# Autodesk Inventor assembly: Wrist
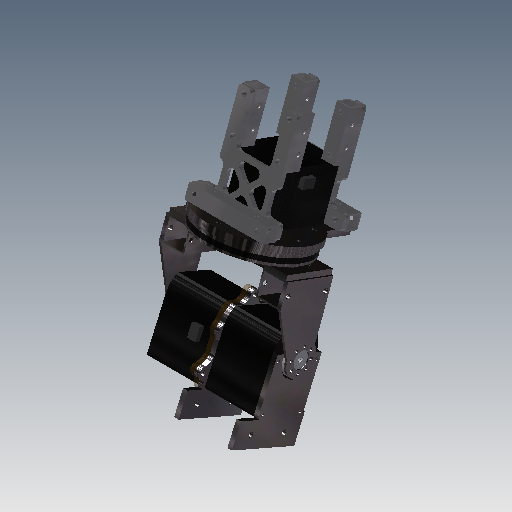
[picture p0: Inventor's stored thumbnail of the model, 512x512]
Saved by Autodesk Inventor 2019.4 (Build 234330000, 330)
## iProperties
Created: 2019-06-30
Part Number: Wrist
Document SubType Name: Assembly
Designer: AzLIer
Author: AzLIer
## Documents named in this file (7)
- E:\ロボ研\キャチロボ\キャチロボ2019\CADdata\アーム2019\Wrist\Wrist.iam
- E:\ロボ研\キャチロボ\キャチロボ2019\CADdata\アーム2019\Wrist\Slide_2_ver2.iam
- E:\ロボ研\キャチロボ\キャチロボ2019\CADdata\アーム2019\Wrist\肩ピッチユニット固定角柱A_9×9.ipt
- E:\ロボ研\キャチロボ\キャチロボ2019\CADdata\アーム2019\Wrist\肩ピッチ固定板_アルミ(A2017)_t3.ipt
- E:\ロボ研\キャチロボ\キャチロボ2019\CADdata\アーム2019\Wrist\肩ピッチ固定角柱B_9×9.ipt
- E:\ロボ研\キャチロボ\キャチロボ2019\CADdata\アーム2019\Wrist\手首関節.iam
- E:\ロボ研\キャチロボ\キャチロボ2019\CADdata\アーム2019\Wrist\先端アームパーツA.ipt
## Components (11 placed, 6 different names)
1. Slide_2:1 [sub-assembly] — 回転:2
2. 肩ピッチユニット固定角柱A_9×9:1
3. 肩ピッチユニット固定角柱A_9×9:2
4. 肩ピッチ固定板_アルミ(A2017)_t3:1
5. 肩ピッチ固定板_アルミ(A2017)_t3:2
6. 肩ピッチ固定角柱B_9×9:1
7. 肩ピッチ固定角柱B_9×9:2
8. 肩ピッチ固定角柱B_9×9:3
9. 肩ピッチ固定角柱B_9×9:4
10. 手首関節:1 [sub-assembly] — 回転:1
11. 先端アームパーツA:1 — 回転:1, 回転:2
## Relationships (26: Mate 22, Flush 2, RevoluteJoint 2)
- [Mate]: Slide_2:1 ↔ 肩ピッチユニット固定角柱A_9×9:1
- [Flush] (10 mm): Slide_2:1 ↔ 肩ピッチユニット固定角柱A_9×9:1
- [Mate] (3 mm): Slide_2:1 ↔ 肩ピッチユニット固定角柱A_9×9:1
- [Mate]: Slide_2:1 ↔ 肩ピッチユニット固定角柱A_9×9:2
- [Flush] (10 mm): Slide_2:1 ↔ 肩ピッチユニット固定角柱A_9×9:2
- [Mate] (3 mm): Slide_2:1 ↔ 肩ピッチユニット固定角柱A_9×9:2
- [Mate]: 肩ピッチユニット固定角柱A_9×9:1 ↔ 肩ピッチ固定板_アルミ(A2017)_t3:1
- [Mate]: 肩ピッチユニット固定角柱A_9×9:1 ↔ 肩ピッチ固定板_アルミ(A2017)_t3:1
- [Mate]: 肩ピッチユニット固定角柱A_9×9:1 ↔ 肩ピッチ固定板_アルミ(A2017)_t3:1
- [Mate]: Slide_2:1 ↔ 肩ピッチ固定板_アルミ(A2017)_t3:2
- [Mate]: 肩ピッチユニット固定角柱A_9×9:2 ↔ 肩ピッチ固定板_アルミ(A2017)_t3:2
- [Mate]: 肩ピッチユニット固定角柱A_9×9:2 ↔ 肩ピッチ固定板_アルミ(A2017)_t3:2
- [Mate]: 肩ピッチ固定板_アルミ(A2017)_t3:1 ↔ 肩ピッチ固定角柱B_9×9:1
- [Mate]: 肩ピッチ固定板_アルミ(A2017)_t3:1 ↔ 肩ピッチ固定角柱B_9×9:1
- [Mate]: 肩ピッチ固定板_アルミ(A2017)_t3:1 ↔ 肩ピッチ固定角柱B_9×9:1
- [Mate]: 肩ピッチ固定板_アルミ(A2017)_t3:2 ↔ 肩ピッチ固定角柱B_9×9:2
- [Mate]: 肩ピッチ固定板_アルミ(A2017)_t3:2 ↔ 肩ピッチ固定角柱B_9×9:2
- [Mate]: 肩ピッチ固定板_アルミ(A2017)_t3:2 ↔ 肩ピッチ固定角柱B_9×9:2
- [Mate]: 肩ピッチ固定板_アルミ(A2017)_t3:1 ↔ 肩ピッチ固定角柱B_9×9:4
- [Mate]: 肩ピッチ固定板_アルミ(A2017)_t3:2 ↔ 肩ピッチ固定角柱B_9×9:3
- [Mate]: 肩ピッチ固定板_アルミ(A2017)_t3:1 ↔ 肩ピッチ固定角柱B_9×9:4
- [Mate]: 肩ピッチ固定板_アルミ(A2017)_t3:1 ↔ 肩ピッチ固定角柱B_9×9:4
- [Mate]: 肩ピッチ固定板_アルミ(A2017)_t3:2 ↔ 肩ピッチ固定角柱B_9×9:3
- [Mate]: 肩ピッチ固定板_アルミ(A2017)_t3:2 ↔ 肩ピッチ固定角柱B_9×9:3
- 回転:1 [RevoluteJoint]: 手首関節:1 ↔ 先端アームパーツA:1
- 回転:2 [RevoluteJoint]: Slide_2:1 ↔ 先端アームパーツA:1
